# Autodesk Inventor assembly: z_mount_assembly
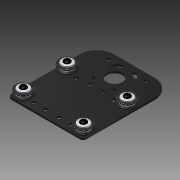
[picture p0: Inventor's stored thumbnail of the model, 180x180]
Saved by Autodesk Inventor 2014 (Build 180170000, 170)
## iProperties
Created: 2013-07-18
Part Number: z_mount_assembly
Document SubType Name: Assembly
Designer: Edward
Author: Edward
## Documents named in this file (7)
- C:\Users\Edward\Desktop\Shapeoko_v2.0\shapeoko_lowpro\z_mount_assembly.iam
- C:\Users\Edward\Desktop\Shapeoko_v2.0\shapeoko_lowpro\x_motor_mount_v2.ipt
- C:\Users\Edward\Desktop\Shapeoko_v2.0\B30037.iam
- C:\Users\Edward\Desktop\Shapeoko_v2.0\SM-H03.ipt
- C:\Users\Edward\Desktop\Shapeoko_v2.0\91239A233.ipt
- C:\Users\Edward\Desktop\Shapeoko_v2.0\SM-H04.ipt
- C:\Users\Edward\Desktop\Shapeoko_v2.0\B18033.ipt
## Components (19 placed, 6 different names)
1. x_motor_mount_v2:1 — Insert:7, Insert:8, Insert:9, Insert:10, Insert:13, Insert:16, Mate:3, Mate:4
2. B30037:1 [sub-assembly]
3. SM-H03:1 — Insert:7
4. 91239A233:1
5. SM-H04:1
6. SM-H03:2 — Insert:9
7. B30037:2 [sub-assembly]
8. SM-H03:3 — Insert:8
9. 91239A233:2
10. SM-H04:2
11. SM-H03:4 — Insert:10
12. B18033:1 — Insert:13
13. SM-H03:5 — Mate:4
14. 91239A233:3
15. B30037:3 [sub-assembly]
16. B18033:2 — Insert:16
17. SM-H03:6 — Mate:3
18. 91239A233:4
19. B30037:4 [sub-assembly]
## Relationships (20: Insert 16, Mate 4)
- [Insert]: B30037:1 ↔ SM-H03:1
- [Insert]: B30037:1 ↔ 91239A233:1
- [Insert]: SM-H04:1 ↔ SM-H03:2
- [Insert]: B30037:2 ↔ SM-H03:3
- [Insert]: B30037:2 ↔ 91239A233:2
- [Insert]: SM-H04:2 ↔ SM-H03:4
- Insert:7: x_motor_mount_v2:1 ↔ SM-H03:1
- Insert:8: x_motor_mount_v2:1 ↔ SM-H03:3
- Insert:9: x_motor_mount_v2:1 ↔ SM-H03:2
- Insert:10: x_motor_mount_v2:1 ↔ SM-H03:4
- [Insert]: SM-H03:5 ↔ B30037:3
- [Insert]: 91239A233:3 ↔ B30037:3
- [Mate]: B18033:1 ↔ 91239A233:3
- Insert:13: x_motor_mount_v2:1 ↔ B18033:1
- [Insert]: SM-H03:6 ↔ B30037:4
- [Insert]: 91239A233:4 ↔ B30037:4
- [Mate]: B18033:2 ↔ 91239A233:4
- Insert:16: x_motor_mount_v2:1 ↔ B18033:2
- Mate:3: x_motor_mount_v2:1 ↔ SM-H03:6
- Mate:4: x_motor_mount_v2:1 ↔ SM-H03:5
## Named parameters: d17_d1 = 0 mm, d18_d7 = 0 mm, d3_d17_d1 = 0 mm, d4_d18_d7 = 0 mm, d5_d9 = 0 mm, d11_d10 = 0 mm, d22_d12 = 0 mm, d15_d10 = 0 mm, d16_d11 = 0 mm, d17_d22_d12 = 0 mm
